# Autodesk Inventor assembly: zlozenie_kompetne_WIZUAL2
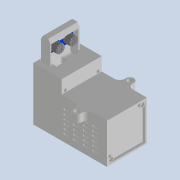
[picture p0: Inventor's stored thumbnail of the model, 180x180]
Saved by Autodesk Inventor 2021 (Build 250183000, 183)
## iProperties
Created: 2025-11-29
Part Number: zlozenie_kompetne_WIZUAL2
Document SubType Name: Assembly
Designer: huber
Author: huber
## Documents named in this file (5)
- C:\Users\huber\OneDrive\Pulpit\hackaton BHL\BHL 2025\zlozenie_kompetne_WIZUAL2.iam
- C:\Users\huber\OneDrive\Pulpit\hackaton BHL\BHL 2025\pokrywa_obudowa.ipt
- C:\Users\huber\OneDrive\Pulpit\hackaton BHL\BHL 2025\Drawer.iam
- C:\Users\huber\OneDrive\Pulpit\hackaton BHL\BHL 2025\obudowa_WIZ2.ipt
- C:\Users\huber\Downloads\Solar Panel.ipt
## Components (4 placed, 4 different names)
1. pokrywa_obudowa:1 — Insert:1
2. Drawer:1 [sub-assembly] — Flush:1, Flush:2, Mate:1, Flush:3, Mate:2, Mate:3
3. obudowa_WIZ2:1 — Flush:1, Flush:2, Mate:1, Insert:1
4. Solar Panel:1 — Flush:3, Mate:2, Mate:3
## Relationships (7: Flush 3, Mate 3, Insert 1)
- Flush:1: Drawer:1 ↔ obudowa_WIZ2:1
- Flush:2: Drawer:1 ↔ obudowa_WIZ2:1
- Mate:1: Drawer:1 ↔ obudowa_WIZ2:1
- Insert:1: pokrywa_obudowa:1 ↔ obudowa_WIZ2:1
- Flush:3 (4.375 mm): Drawer:1 ↔ Solar Panel:1
- Mate:2: Drawer:1 ↔ Solar Panel:1
- Mate:3: Drawer:1 ↔ Solar Panel:1
